# Autodesk Inventor assembly: SmartTrash Tinggi
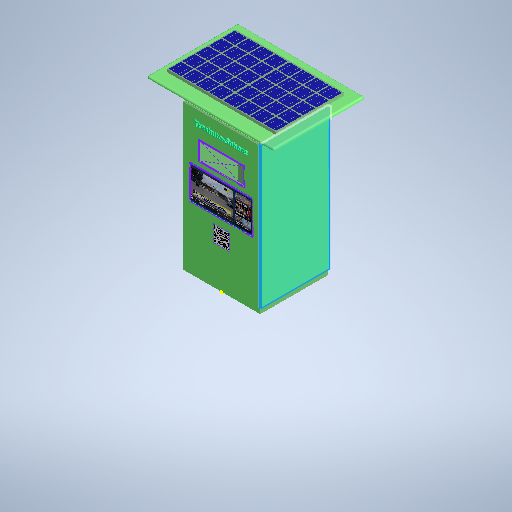
[picture p0: Inventor's stored thumbnail of the model, 512x512]
Saved by Autodesk Inventor 2025.2 (Build 292293000, 293)
## iProperties
Created: 2025-04-04
Part Number: SmartTrash Tinggi
Document SubType Name: Assembly
Designer: hando
Author: hando
## Documents named in this file (13)
- D:\Data_Lokal\Kuliah\Tri Wahyu (22518241023)\Lomba Essay\Himepa\SmartTrash\SmartTrash Tinggi.iam
- D:\Data_Lokal\Kuliah\Tri Wahyu (22518241023)\Lomba Essay\Himepa\SmartTrash\TempatSampahTinggi.ipt
- D:\Data_Lokal\Kuliah\Tri Wahyu (22518241023)\Lomba Essay\Himepa\SmartTrash\Solar panel.ipt
- D:\Data_Lokal\Kuliah\Tri Wahyu (22518241023)\Lomba Essay\Himepa\SmartTrash\TutupAtasTP.ipt
- D:\Data_Lokal\Kuliah\Tri Wahyu (22518241023)\Lomba Essay\Himepa\SmartTrash\TutupSampingTP.ipt
- D:\Data_Lokal\Kuliah\Tri Wahyu (22518241023)\Lomba Essay\Himepa\SmartTrash\Raspi5.ipt
- D:\Data_Lokal\Kuliah\Tri Wahyu (22518241023)\Lomba Essay\Himepa\logitech-c270-webcam-1.snapshot.1\Logitech c270 Assembly\Logitech c270 Assembly\Logitech c270 Assembly.iam
- D:\Data_Lokal\Kuliah\Tri Wahyu (22518241023)\Lomba Essay\Himepa\linear-drive-the-xy-axes-1.snapshot.2\лінійн-перемXY\лінійн-перемXY\лінійн-перемXY.iam
- D:\Data_Lokal\Kuliah\Tri Wahyu (22518241023)\Lomba Essay\Himepa\SmartTrash\SorterTP.ipt
- D:\Data_Lokal\Kuliah\Tri Wahyu (22518241023)\Lomba Essay\Himepa\SmartTrash\FinalAssembly.iam
- D:\Data_Lokal\Kuliah\Tri Wahyu (22518241023)\Lomba Essay\Himepa\SmartTrash\driverbtn v1.iam
- D:\Data_Lokal\Kuliah\Tri Wahyu (22518241023)\Lomba Essay\Himepa\SmartTrash\BATERIA.ipt
- D:\Data_Lokal\Kuliah\Tri Wahyu (22518241023)\Lomba Essay\Himepa\SmartTrash\LoadCell besar.ipt
## Components (14 placed, 12 different names)
1. TempatSampahTinggi:1 — Mate:2, Mate:3, Mate:4, Mate:8, Mate:12, Mate:14, Flush:5, Mate:16
2. Solar panel:1 — Mate:1, Flush:1, Flush:2, Mate:10
3. Solar panel:2 — Mate:1, Flush:1, Flush:2, Mate:5, Mate:9
4. TutupAtasTP:1 — Mate:2, Mate:5, Mate:6, Mate:7, Mate:8, Mate:9, Mate:10, Flush:3, Flush:4, Mate:11, Mate:17, Mate:18, Flush:6, Flush:7, Mate:19
5. TutupSampingTP:1 — Mate:3, Mate:4
6. Raspi5:1 — Mate:6, Flush:3, Flush:4
7. Logitech c270 Assembly:1 [sub-assembly] — Mate:7, Mate:11
8. лінійн-перемXY:1 [sub-assembly] — Mate:12, Mate:13, Mate:14, Flush:5, Mate:15
9. SorterTP:1 — Mate:13, Mate:15
10. FinalAssembly:1 [sub-assembly] — Mate:16, Mate:20
11. driverbtn v1:1 [sub-assembly] — Mate:17, Flush:6
12. driverbtn v1:2 [sub-assembly] — Mate:18, Flush:7
13. BATERIA:1 — Mate:19
14. LoadCell besar:1 — Mate:20
## Relationships (27: Mate 20, Flush 7)
- Mate:1: Solar panel:1 ↔ Solar panel:2
- Flush:1: Solar panel:1 ↔ Solar panel:2
- Flush:2: Solar panel:1 ↔ Solar panel:2
- Mate:2: TempatSampahTinggi:1 ↔ TutupAtasTP:1
- Mate:3: TempatSampahTinggi:1 ↔ TutupSampingTP:1
- Mate:4: TempatSampahTinggi:1 ↔ TutupSampingTP:1
- Mate:5: Solar panel:2 ↔ TutupAtasTP:1
- Mate:6: TutupAtasTP:1 ↔ Raspi5:1
- Mate:7: TutupAtasTP:1 ↔ Logitech c270 Assembly:1
- Mate:8 (-20 mm): TempatSampahTinggi:1 ↔ TutupAtasTP:1
- Mate:9 (60 mm): Solar panel:2 ↔ TutupAtasTP:1
- Mate:10 (140 mm): Solar panel:1 ↔ TutupAtasTP:1
- Flush:3 (200 mm): TutupAtasTP:1 ↔ Raspi5:1
- Flush:4 (300 mm): TutupAtasTP:1 ↔ Raspi5:1
- Mate:11: TutupAtasTP:1 ↔ Logitech c270 Assembly:1
- Mate:12: TempatSampahTinggi:1 ↔ лінійн-перемXY:1
- Mate:13: лінійн-перемXY:1 ↔ SorterTP:1
- Mate:14 (100 mm): TempatSampahTinggi:1 ↔ лінійн-перемXY:1
- Flush:5 (50 mm): TempatSampahTinggi:1 ↔ лінійн-перемXY:1
- Mate:15: лінійн-перемXY:1 ↔ SorterTP:1
- Mate:16: TempatSampahTinggi:1 ↔ FinalAssembly:1
- Mate:17: TutupAtasTP:1 ↔ driverbtn v1:1
- Mate:18: TutupAtasTP:1 ↔ driverbtn v1:2
- Flush:6: TutupAtasTP:1 ↔ driverbtn v1:1
- Flush:7: TutupAtasTP:1 ↔ driverbtn v1:2
- Mate:19: TutupAtasTP:1 ↔ BATERIA:1
- Mate:20: FinalAssembly:1 ↔ LoadCell besar:1
